(part 1 of 3)
# Autodesk Inventor assembly: Assembly
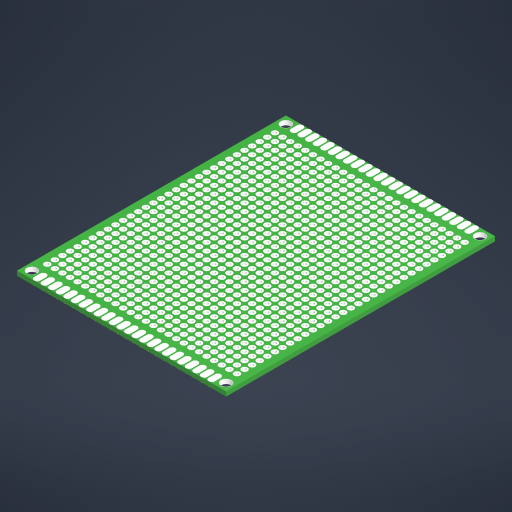
[picture p0: Inventor's stored thumbnail of the model, 512x512]
Saved by Autodesk Inventor 2024 (Build 280153000, 153)
## iProperties
Created: 2024-02-01
Part Number: Assembly
Document SubType Name: Assembly
Designer: Vincent Larson
Title: Universal_board_70x90mm_31x26.stp
Preprocessor: spGate 19.8.4 (****-****-****-****)
## Documents named in this file (908)
- C:\Users\Vincent Larson\Downloads\Universal_board_70x90mm_31x26\Universal_board_70x90mm_31x26.iam
- C:\Users\Vincent Larson\Downloads\Universal_board_70x90mm_31x26\Universal_board_70x90mm_31x26-prt0.ipt
- C:\Users\Vincent Larson\Downloads\Universal_board_70x90mm_31x26\Universal_board_70x90mm_31x26-prt1.ipt
- C:\Users\Vincent Larson\Downloads\Universal_board_70x90mm_31x26\Universal_board_70x90mm_31x26-prt2.ipt
- C:\Users\Vincent Larson\Downloads\Universal_board_70x90mm_31x26\Universal_board_70x90mm_31x26-prt3.ipt
- C:\Users\Vincent Larson\Downloads\Universal_board_70x90mm_31x26\Universal_board_70x90mm_31x26-prt4.ipt
- C:\Users\Vincent Larson\Downloads\Universal_board_70x90mm_31x26\Universal_board_70x90mm_31x26-prt5.ipt
- C:\Users\Vincent Larson\Downloads\Universal_board_70x90mm_31x26\Universal_board_70x90mm_31x26-prt6.ipt
- C:\Users\Vincent Larson\Downloads\Universal_board_70x90mm_31x26\Universal_board_70x90mm_31x26-prt7.ipt
- C:\Users\Vincent Larson\Downloads\Universal_board_70x90mm_31x26\Universal_board_70x90mm_31x26-prt8.ipt
- C:\Users\Vincent Larson\Downloads\Universal_board_70x90mm_31x26\Universal_board_70x90mm_31x26-prt9.ipt
- C:\Users\Vincent Larson\Downloads\Universal_board_70x90mm_31x26\Universal_board_70x90mm_31x26-prt10.ipt
- C:\Users\Vincent Larson\Downloads\Universal_board_70x90mm_31x26\Universal_board_70x90mm_31x26-prt11.ipt
- C:\Users\Vincent Larson\Downloads\Universal_board_70x90mm_31x26\Universal_board_70x90mm_31x26-prt12.ipt
- C:\Users\Vincent Larson\Downloads\Universal_board_70x90mm_31x26\Universal_board_70x90mm_31x26-prt13.ipt
- C:\Users\Vincent Larson\Downloads\Universal_board_70x90mm_31x26\Universal_board_70x90mm_31x26-prt14.ipt
- C:\Users\Vincent Larson\Downloads\Universal_board_70x90mm_31x26\Universal_board_70x90mm_31x26-prt15.ipt
- C:\Users\Vincent Larson\Downloads\Universal_board_70x90mm_31x26\Universal_board_70x90mm_31x26-prt16.ipt
- C:\Users\Vincent Larson\Downloads\Universal_board_70x90mm_31x26\Universal_board_70x90mm_31x26-prt17.ipt
- C:\Users\Vincent Larson\Downloads\Universal_board_70x90mm_31x26\Universal_board_70x90mm_31x26-prt18.ipt
- C:\Users\Vincent Larson\Downloads\Universal_board_70x90mm_31x26\Universal_board_70x90mm_31x26-prt19.ipt
- C:\Users\Vincent Larson\Downloads\Universal_board_70x90mm_31x26\Universal_board_70x90mm_31x26-prt20.ipt
- C:\Users\Vincent Larson\Downloads\Universal_board_70x90mm_31x26\Universal_board_70x90mm_31x26-prt21.ipt
- C:\Users\Vincent Larson\Downloads\Universal_board_70x90mm_31x26\Universal_board_70x90mm_31x26-prt22.ipt
- C:\Users\Vincent Larson\Downloads\Universal_board_70x90mm_31x26\Universal_board_70x90mm_31x26-prt23.ipt
- C:\Users\Vincent Larson\Downloads\Universal_board_70x90mm_31x26\Universal_board_70x90mm_31x26-prt24.ipt
- C:\Users\Vincent Larson\Downloads\Universal_board_70x90mm_31x26\Universal_board_70x90mm_31x26-prt25.ipt
- C:\Users\Vincent Larson\Downloads\Universal_board_70x90mm_31x26\Universal_board_70x90mm_31x26-prt26.ipt
- C:\Users\Vincent Larson\Downloads\Universal_board_70x90mm_31x26\Universal_board_70x90mm_31x26-prt27.ipt
- C:\Users\Vincent Larson\Downloads\Universal_board_70x90mm_31x26\Universal_board_70x90mm_31x26-prt28.ipt
- C:\Users\Vincent Larson\Downloads\Universal_board_70x90mm_31x26\Universal_board_70x90mm_31x26-prt29.ipt
- C:\Users\Vincent Larson\Downloads\Universal_board_70x90mm_31x26\Universal_board_70x90mm_31x26-prt30.ipt
- C:\Users\Vincent Larson\Downloads\Universal_board_70x90mm_31x26\Universal_board_70x90mm_31x26-prt31.ipt
- C:\Users\Vincent Larson\Downloads\Universal_board_70x90mm_31x26\Universal_board_70x90mm_31x26-prt32.ipt
- C:\Users\Vincent Larson\Downloads\Universal_board_70x90mm_31x26\Universal_board_70x90mm_31x26-prt33.ipt
- C:\Users\Vincent Larson\Downloads\Universal_board_70x90mm_31x26\Universal_board_70x90mm_31x26-prt34.ipt
- C:\Users\Vincent Larson\Downloads\Universal_board_70x90mm_31x26\Universal_board_70x90mm_31x26-prt35.ipt
- C:\Users\Vincent Larson\Downloads\Universal_board_70x90mm_31x26\Universal_board_70x90mm_31x26-prt36.ipt
- C:\Users\Vincent Larson\Downloads\Universal_board_70x90mm_31x26\Universal_board_70x90mm_31x26-prt37.ipt
- C:\Users\Vincent Larson\Downloads\Universal_board_70x90mm_31x26\Universal_board_70x90mm_31x26-prt38.ipt
- C:\Users\Vincent Larson\Downloads\Universal_board_70x90mm_31x26\Universal_board_70x90mm_31x26-prt39.ipt
- C:\Users\Vincent Larson\Downloads\Universal_board_70x90mm_31x26\Universal_board_70x90mm_31x26-prt40.ipt
- C:\Users\Vincent Larson\Downloads\Universal_board_70x90mm_31x26\Universal_board_70x90mm_31x26-prt41.ipt
- C:\Users\Vincent Larson\Downloads\Universal_board_70x90mm_31x26\Universal_board_70x90mm_31x26-prt42.ipt
- C:\Users\Vincent Larson\Downloads\Universal_board_70x90mm_31x26\Universal_board_70x90mm_31x26-prt43.ipt
- C:\Users\Vincent Larson\Downloads\Universal_board_70x90mm_31x26\Universal_board_70x90mm_31x26-prt44.ipt
- C:\Users\Vincent Larson\Downloads\Universal_board_70x90mm_31x26\Universal_board_70x90mm_31x26-prt45.ipt
- C:\Users\Vincent Larson\Downloads\Universal_board_70x90mm_31x26\Universal_board_70x90mm_31x26-prt46.ipt
- C:\Users\Vincent Larson\Downloads\Universal_board_70x90mm_31x26\Universal_board_70x90mm_31x26-prt47.ipt
- C:\Users\Vincent Larson\Downloads\Universal_board_70x90mm_31x26\Universal_board_70x90mm_31x26-prt48.ipt
- C:\Users\Vincent Larson\Downloads\Universal_board_70x90mm_31x26\Universal_board_70x90mm_31x26-prt49.ipt
- C:\Users\Vincent Larson\Downloads\Universal_board_70x90mm_31x26\Universal_board_70x90mm_31x26-prt50.ipt
- C:\Users\Vincent Larson\Downloads\Universal_board_70x90mm_31x26\Universal_board_70x90mm_31x26-prt51.ipt
- C:\Users\Vincent Larson\Downloads\Universal_board_70x90mm_31x26\Universal_board_70x90mm_31x26-prt52.ipt
- C:\Users\Vincent Larson\Downloads\Universal_board_70x90mm_31x26\Universal_board_70x90mm_31x26-prt53.ipt
- C:\Users\Vincent Larson\Downloads\Universal_board_70x90mm_31x26\Universal_board_70x90mm_31x26-prt54.ipt
- C:\Users\Vincent Larson\Downloads\Universal_board_70x90mm_31x26\Universal_board_70x90mm_31x26-prt55.ipt
- C:\Users\Vincent Larson\Downloads\Universal_board_70x90mm_31x26\Universal_board_70x90mm_31x26-prt56.ipt
- C:\Users\Vincent Larson\Downloads\Universal_board_70x90mm_31x26\Universal_board_70x90mm_31x26-prt57.ipt
- C:\Users\Vincent Larson\Downloads\Universal_board_70x90mm_31x26\Universal_board_70x90mm_31x26-prt58.ipt
- C:\Users\Vincent Larson\Downloads\Universal_board_70x90mm_31x26\Universal_board_70x90mm_31x26-prt59.ipt
- C:\Users\Vincent Larson\Downloads\Universal_board_70x90mm_31x26\Universal_board_70x90mm_31x26-prt60.ipt
- C:\Users\Vincent Larson\Downloads\Universal_board_70x90mm_31x26\Universal_board_70x90mm_31x26-prt61.ipt
- C:\Users\Vincent Larson\Downloads\Universal_board_70x90mm_31x26\Universal_board_70x90mm_31x26-prt62.ipt
- C:\Users\Vincent Larson\Downloads\Universal_board_70x90mm_31x26\Universal_board_70x90mm_31x26-prt63.ipt
- C:\Users\Vincent Larson\Downloads\Universal_board_70x90mm_31x26\Universal_board_70x90mm_31x26-prt64.ipt
- C:\Users\Vincent Larson\Downloads\Universal_board_70x90mm_31x26\Universal_board_70x90mm_31x26-prt65.ipt
- C:\Users\Vincent Larson\Downloads\Universal_board_70x90mm_31x26\Universal_board_70x90mm_31x26-prt66.ipt
- C:\Users\Vincent Larson\Downloads\Universal_board_70x90mm_31x26\Universal_board_70x90mm_31x26-prt67.ipt
- C:\Users\Vincent Larson\Downloads\Universal_board_70x90mm_31x26\Universal_board_70x90mm_31x26-prt68.ipt
- C:\Users\Vincent Larson\Downloads\Universal_board_70x90mm_31x26\Universal_board_70x90mm_31x26-prt69.ipt
- C:\Users\Vincent Larson\Downloads\Universal_board_70x90mm_31x26\Universal_board_70x90mm_31x26-prt70.ipt
- C:\Users\Vincent Larson\Downloads\Universal_board_70x90mm_31x26\Universal_board_70x90mm_31x26-prt71.ipt
- C:\Users\Vincent Larson\Downloads\Universal_board_70x90mm_31x26\Universal_board_70x90mm_31x26-prt72.ipt
- C:\Users\Vincent Larson\Downloads\Universal_board_70x90mm_31x26\Universal_board_70x90mm_31x26-prt73.ipt
- C:\Users\Vincent Larson\Downloads\Universal_board_70x90mm_31x26\Universal_board_70x90mm_31x26-prt74.ipt
- C:\Users\Vincent Larson\Downloads\Universal_board_70x90mm_31x26\Universal_board_70x90mm_31x26-prt75.ipt
- C:\Users\Vincent Larson\Downloads\Universal_board_70x90mm_31x26\Universal_board_70x90mm_31x26-prt76.ipt
- C:\Users\Vincent Larson\Downloads\Universal_board_70x90mm_31x26\Universal_board_70x90mm_31x26-prt77.ipt
- C:\Users\Vincent Larson\Downloads\Universal_board_70x90mm_31x26\Universal_board_70x90mm_31x26-prt78.ipt
- C:\Users\Vincent Larson\Downloads\Universal_board_70x90mm_31x26\Universal_board_70x90mm_31x26-prt79.ipt
- C:\Users\Vincent Larson\Downloads\Universal_board_70x90mm_31x26\Universal_board_70x90mm_31x26-prt80.ipt
- C:\Users\Vincent Larson\Downloads\Universal_board_70x90mm_31x26\Universal_board_70x90mm_31x26-prt81.ipt
- C:\Users\Vincent Larson\Downloads\Universal_board_70x90mm_31x26\Universal_board_70x90mm_31x26-prt82.ipt
- C:\Users\Vincent Larson\Downloads\Universal_board_70x90mm_31x26\Universal_board_70x90mm_31x26-prt83.ipt
- C:\Users\Vincent Larson\Downloads\Universal_board_70x90mm_31x26\Universal_board_70x90mm_31x26-prt84.ipt
- C:\Users\Vincent Larson\Downloads\Universal_board_70x90mm_31x26\Universal_board_70x90mm_31x26-prt85.ipt
- C:\Users\Vincent Larson\Downloads\Universal_board_70x90mm_31x26\Universal_board_70x90mm_31x26-prt86.ipt
- C:\Users\Vincent Larson\Downloads\Universal_board_70x90mm_31x26\Universal_board_70x90mm_31x26-prt87.ipt
- C:\Users\Vincent Larson\Downloads\Universal_board_70x90mm_31x26\Universal_board_70x90mm_31x26-prt88.ipt
- C:\Users\Vincent Larson\Downloads\Universal_board_70x90mm_31x26\Universal_board_70x90mm_31x26-prt89.ipt
- C:\Users\Vincent Larson\Downloads\Universal_board_70x90mm_31x26\Universal_board_70x90mm_31x26-prt90.ipt
- C:\Users\Vincent Larson\Downloads\Universal_board_70x90mm_31x26\Universal_board_70x90mm_31x26-prt91.ipt
- C:\Users\Vincent Larson\Downloads\Universal_board_70x90mm_31x26\Universal_board_70x90mm_31x26-prt92.ipt
- C:\Users\Vincent Larson\Downloads\Universal_board_70x90mm_31x26\Universal_board_70x90mm_31x26-prt93.ipt
- C:\Users\Vincent Larson\Downloads\Universal_board_70x90mm_31x26\Universal_board_70x90mm_31x26-prt94.ipt
- C:\Users\Vincent Larson\Downloads\Universal_board_70x90mm_31x26\Universal_board_70x90mm_31x26-prt95.ipt
- C:\Users\Vincent Larson\Downloads\Universal_board_70x90mm_31x26\Universal_board_70x90mm_31x26-prt96.ipt
- C:\Users\Vincent Larson\Downloads\Universal_board_70x90mm_31x26\Universal_board_70x90mm_31x26-prt97.ipt
- C:\Users\Vincent Larson\Downloads\Universal_board_70x90mm_31x26\Universal_board_70x90mm_31x26-prt98.ipt
- C:\Users\Vincent Larson\Downloads\Universal_board_70x90mm_31x26\Universal_board_70x90mm_31x26-prt99.ipt
- C:\Users\Vincent Larson\Downloads\Universal_board_70x90mm_31x26\Universal_board_70x90mm_31x26-prt100.ipt
- C:\Users\Vincent Larson\Downloads\Universal_board_70x90mm_31x26\Universal_board_70x90mm_31x26-prt101.ipt
- C:\Users\Vincent Larson\Downloads\Universal_board_70x90mm_31x26\Universal_board_70x90mm_31x26-prt102.ipt
- C:\Users\Vincent Larson\Downloads\Universal_board_70x90mm_31x26\Universal_board_70x90mm_31x26-prt103.ipt
- C:\Users\Vincent Larson\Downloads\Universal_board_70x90mm_31x26\Universal_board_70x90mm_31x26-prt104.ipt
- C:\Users\Vincent Larson\Downloads\Universal_board_70x90mm_31x26\Universal_board_70x90mm_31x26-prt105.ipt
- C:\Users\Vincent Larson\Downloads\Universal_board_70x90mm_31x26\Universal_board_70x90mm_31x26-prt106.ipt
- C:\Users\Vincent Larson\Downloads\Universal_board_70x90mm_31x26\Universal_board_70x90mm_31x26-prt107.ipt
- C:\Users\Vincent Larson\Downloads\Universal_board_70x90mm_31x26\Universal_board_70x90mm_31x26-prt108.ipt
- C:\Users\Vincent Larson\Downloads\Universal_board_70x90mm_31x26\Universal_board_70x90mm_31x26-prt109.ipt
- C:\Users\Vincent Larson\Downloads\Universal_board_70x90mm_31x26\Universal_board_70x90mm_31x26-prt110.ipt
- C:\Users\Vincent Larson\Downloads\Universal_board_70x90mm_31x26\Universal_board_70x90mm_31x26-prt111.ipt
- C:\Users\Vincent Larson\Downloads\Universal_board_70x90mm_31x26\Universal_board_70x90mm_31x26-prt112.ipt
- C:\Users\Vincent Larson\Downloads\Universal_board_70x90mm_31x26\Universal_board_70x90mm_31x26-prt113.ipt
- C:\Users\Vincent Larson\Downloads\Universal_board_70x90mm_31x26\Universal_board_70x90mm_31x26-prt114.ipt
- C:\Users\Vincent Larson\Downloads\Universal_board_70x90mm_31x26\Universal_board_70x90mm_31x26-prt115.ipt
- C:\Users\Vincent Larson\Downloads\Universal_board_70x90mm_31x26\Universal_board_70x90mm_31x26-prt116.ipt
- C:\Users\Vincent Larson\Downloads\Universal_board_70x90mm_31x26\Universal_board_70x90mm_31x26-prt117.ipt
- C:\Users\Vincent Larson\Downloads\Universal_board_70x90mm_31x26\Universal_board_70x90mm_31x26-prt118.ipt
- C:\Users\Vincent Larson\Downloads\Universal_board_70x90mm_31x26\Universal_board_70x90mm_31x26-prt119.ipt
- C:\Users\Vincent Larson\Downloads\Universal_board_70x90mm_31x26\Universal_board_70x90mm_31x26-prt120.ipt
- C:\Users\Vincent Larson\Downloads\Universal_board_70x90mm_31x26\Universal_board_70x90mm_31x26-prt121.ipt
- C:\Users\Vincent Larson\Downloads\Universal_board_70x90mm_31x26\Universal_board_70x90mm_31x26-prt122.ipt
- C:\Users\Vincent Larson\Downloads\Universal_board_70x90mm_31x26\Universal_board_70x90mm_31x26-prt123.ipt
- C:\Users\Vincent Larson\Downloads\Universal_board_70x90mm_31x26\Universal_board_70x90mm_31x26-prt124.ipt
- C:\Users\Vincent Larson\Downloads\Universal_board_70x90mm_31x26\Universal_board_70x90mm_31x26-prt125.ipt
- C:\Users\Vincent Larson\Downloads\Universal_board_70x90mm_31x26\Universal_board_70x90mm_31x26-prt126.ipt
- C:\Users\Vincent Larson\Downloads\Universal_board_70x90mm_31x26\Universal_board_70x90mm_31x26-prt127.ipt
- C:\Users\Vincent Larson\Downloads\Universal_board_70x90mm_31x26\Universal_board_70x90mm_31x26-prt128.ipt
- C:\Users\Vincent Larson\Downloads\Universal_board_70x90mm_31x26\Universal_board_70x90mm_31x26-prt129.ipt
- C:\Users\Vincent Larson\Downloads\Universal_board_70x90mm_31x26\Universal_board_70x90mm_31x26-prt130.ipt
- C:\Users\Vincent Larson\Downloads\Universal_board_70x90mm_31x26\Universal_board_70x90mm_31x26-prt131.ipt
- C:\Users\Vincent Larson\Downloads\Universal_board_70x90mm_31x26\Universal_board_70x90mm_31x26-prt132.ipt
- C:\Users\Vincent Larson\Downloads\Universal_board_70x90mm_31x26\Universal_board_70x90mm_31x26-prt133.ipt
- C:\Users\Vincent Larson\Downloads\Universal_board_70x90mm_31x26\Universal_board_70x90mm_31x26-prt134.ipt
- C:\Users\Vincent Larson\Downloads\Universal_board_70x90mm_31x26\Universal_board_70x90mm_31x26-prt135.ipt
- C:\Users\Vincent Larson\Downloads\Universal_board_70x90mm_31x26\Universal_board_70x90mm_31x26-prt136.ipt
- C:\Users\Vincent Larson\Downloads\Universal_board_70x90mm_31x26\Universal_board_70x90mm_31x26-prt137.ipt
- C:\Users\Vincent Larson\Downloads\Universal_board_70x90mm_31x26\Universal_board_70x90mm_31x26-prt138.ipt
- C:\Users\Vincent Larson\Downloads\Universal_board_70x90mm_31x26\Universal_board_70x90mm_31x26-prt139.ipt
- C:\Users\Vincent Larson\Downloads\Universal_board_70x90mm_31x26\Universal_board_70x90mm_31x26-prt140.ipt
- C:\Users\Vincent Larson\Downloads\Universal_board_70x90mm_31x26\Universal_board_70x90mm_31x26-prt141.ipt
- C:\Users\Vincent Larson\Downloads\Universal_board_70x90mm_31x26\Universal_board_70x90mm_31x26-prt142.ipt
- C:\Users\Vincent Larson\Downloads\Universal_board_70x90mm_31x26\Universal_board_70x90mm_31x26-prt143.ipt
- C:\Users\Vincent Larson\Downloads\Universal_board_70x90mm_31x26\Universal_board_70x90mm_31x26-prt144.ipt
- C:\Users\Vincent Larson\Downloads\Universal_board_70x90mm_31x26\Universal_board_70x90mm_31x26-prt145.ipt
- C:\Users\Vincent Larson\Downloads\Universal_board_70x90mm_31x26\Universal_board_70x90mm_31x26-prt146.ipt
- C:\Users\Vincent Larson\Downloads\Universal_board_70x90mm_31x26\Universal_board_70x90mm_31x26-prt147.ipt
- C:\Users\Vincent Larson\Downloads\Universal_board_70x90mm_31x26\Universal_board_70x90mm_31x26-prt148.ipt
- C:\Users\Vincent Larson\Downloads\Universal_board_70x90mm_31x26\Universal_board_70x90mm_31x26-prt149.ipt
- C:\Users\Vincent Larson\Downloads\Universal_board_70x90mm_31x26\Universal_board_70x90mm_31x26-prt150.ipt
- C:\Users\Vincent Larson\Downloads\Universal_board_70x90mm_31x26\Universal_board_70x90mm_31x26-prt151.ipt
- C:\Users\Vincent Larson\Downloads\Universal_board_70x90mm_31x26\Universal_board_70x90mm_31x26-prt152.ipt
- C:\Users\Vincent Larson\Downloads\Universal_board_70x90mm_31x26\Universal_board_70x90mm_31x26-prt153.ipt
- C:\Users\Vincent Larson\Downloads\Universal_board_70x90mm_31x26\Universal_board_70x90mm_31x26-prt154.ipt
- C:\Users\Vincent Larson\Downloads\Universal_board_70x90mm_31x26\Universal_board_70x90mm_31x26-prt155.ipt
- C:\Users\Vincent Larson\Downloads\Universal_board_70x90mm_31x26\Universal_board_70x90mm_31x26-prt156.ipt
- C:\Users\Vincent Larson\Downloads\Universal_board_70x90mm_31x26\Universal_board_70x90mm_31x26-prt157.ipt
- C:\Users\Vincent Larson\Downloads\Universal_board_70x90mm_31x26\Universal_board_70x90mm_31x26-prt158.ipt
- C:\Users\Vincent Larson\Downloads\Universal_board_70x90mm_31x26\Universal_board_70x90mm_31x26-prt159.ipt
- C:\Users\Vincent Larson\Downloads\Universal_board_70x90mm_31x26\Universal_board_70x90mm_31x26-prt160.ipt
- C:\Users\Vincent Larson\Downloads\Universal_board_70x90mm_31x26\Universal_board_70x90mm_31x26-prt161.ipt
- C:\Users\Vincent Larson\Downloads\Universal_board_70x90mm_31x26\Universal_board_70x90mm_31x26-prt162.ipt
- C:\Users\Vincent Larson\Downloads\Universal_board_70x90mm_31x26\Universal_board_70x90mm_31x26-prt163.ipt
- C:\Users\Vincent Larson\Downloads\Universal_board_70x90mm_31x26\Universal_board_70x90mm_31x26-prt164.ipt
- C:\Users\Vincent Larson\Downloads\Universal_board_70x90mm_31x26\Universal_board_70x90mm_31x26-prt165.ipt
- C:\Users\Vincent Larson\Downloads\Universal_board_70x90mm_31x26\Universal_board_70x90mm_31x26-prt166.ipt
- C:\Users\Vincent Larson\Downloads\Universal_board_70x90mm_31x26\Universal_board_70x90mm_31x26-prt167.ipt
- C:\Users\Vincent Larson\Downloads\Universal_board_70x90mm_31x26\Universal_board_70x90mm_31x26-prt168.ipt
- C:\Users\Vincent Larson\Downloads\Universal_board_70x90mm_31x26\Universal_board_70x90mm_31x26-prt169.ipt
- C:\Users\Vincent Larson\Downloads\Universal_board_70x90mm_31x26\Universal_board_70x90mm_31x26-prt170.ipt
- C:\Users\Vincent Larson\Downloads\Universal_board_70x90mm_31x26\Universal_board_70x90mm_31x26-prt171.ipt
- C:\Users\Vincent Larson\Downloads\Universal_board_70x90mm_31x26\Universal_board_70x90mm_31x26-prt172.ipt
- C:\Users\Vincent Larson\Downloads\Universal_board_70x90mm_31x26\Universal_board_70x90mm_31x26-prt173.ipt
- C:\Users\Vincent Larson\Downloads\Universal_board_70x90mm_31x26\Universal_board_70x90mm_31x26-prt174.ipt
- C:\Users\Vincent Larson\Downloads\Universal_board_70x90mm_31x26\Universal_board_70x90mm_31x26-prt175.ipt
- C:\Users\Vincent Larson\Downloads\Universal_board_70x90mm_31x26\Universal_board_70x90mm_31x26-prt176.ipt
- C:\Users\Vincent Larson\Downloads\Universal_board_70x90mm_31x26\Universal_board_70x90mm_31x26-prt177.ipt
- C:\Users\Vincent Larson\Downloads\Universal_board_70x90mm_31x26\Universal_board_70x90mm_31x26-prt178.ipt
- C:\Users\Vincent Larson\Downloads\Universal_board_70x90mm_31x26\Universal_board_70x90mm_31x26-prt179.ipt
- C:\Users\Vincent Larson\Downloads\Universal_board_70x90mm_31x26\Universal_board_70x90mm_31x26-prt180.ipt
- C:\Users\Vincent Larson\Downloads\Universal_board_70x90mm_31x26\Universal_board_70x90mm_31x26-prt181.ipt
- C:\Users\Vincent Larson\Downloads\Universal_board_70x90mm_31x26\Universal_board_70x90mm_31x26-prt182.ipt
- C:\Users\Vincent Larson\Downloads\Universal_board_70x90mm_31x26\Universal_board_70x90mm_31x26-prt183.ipt
- C:\Users\Vincent Larson\Downloads\Universal_board_70x90mm_31x26\Universal_board_70x90mm_31x26-prt184.ipt
- C:\Users\Vincent Larson\Downloads\Universal_board_70x90mm_31x26\Universal_board_70x90mm_31x26-prt185.ipt
- C:\Users\Vincent Larson\Downloads\Universal_board_70x90mm_31x26\Universal_board_70x90mm_31x26-prt186.ipt
- C:\Users\Vincent Larson\Downloads\Universal_board_70x90mm_31x26\Universal_board_70x90mm_31x26-prt187.ipt
- C:\Users\Vincent Larson\Downloads\Universal_board_70x90mm_31x26\Universal_board_70x90mm_31x26-prt188.ipt
- C:\Users\Vincent Larson\Downloads\Universal_board_70x90mm_31x26\Universal_board_70x90mm_31x26-prt189.ipt
- C:\Users\Vincent Larson\Downloads\Universal_board_70x90mm_31x26\Universal_board_70x90mm_31x26-prt190.ipt
- C:\Users\Vincent Larson\Downloads\Universal_board_70x90mm_31x26\Universal_board_70x90mm_31x26-prt191.ipt
- C:\Users\Vincent Larson\Downloads\Universal_board_70x90mm_31x26\Universal_board_70x90mm_31x26-prt192.ipt
- C:\Users\Vincent Larson\Downloads\Universal_board_70x90mm_31x26\Universal_board_70x90mm_31x26-prt193.ipt
- C:\Users\Vincent Larson\Downloads\Universal_board_70x90mm_31x26\Universal_board_70x90mm_31x26-prt194.ipt
- C:\Users\Vincent Larson\Downloads\Universal_board_70x90mm_31x26\Universal_board_70x90mm_31x26-prt195.ipt
- C:\Users\Vincent Larson\Downloads\Universal_board_70x90mm_31x26\Universal_board_70x90mm_31x26-prt196.ipt
- C:\Users\Vincent Larson\Downloads\Universal_board_70x90mm_31x26\Universal_board_70x90mm_31x26-prt197.ipt
- C:\Users\Vincent Larson\Downloads\Universal_board_70x90mm_31x26\Universal_board_70x90mm_31x26-prt198.ipt
- C:\Users\Vincent Larson\Downloads\Universal_board_70x90mm_31x26\Universal_board_70x90mm_31x26-prt199.ipt
- C:\Users\Vincent Larson\Downloads\Universal_board_70x90mm_31x26\Universal_board_70x90mm_31x26-prt200.ipt
- C:\Users\Vincent Larson\Downloads\Universal_board_70x90mm_31x26\Universal_board_70x90mm_31x26-prt201.ipt
- C:\Users\Vincent Larson\Downloads\Universal_board_70x90mm_31x26\Universal_board_70x90mm_31x26-prt202.ipt
- C:\Users\Vincent Larson\Downloads\Universal_board_70x90mm_31x26\Universal_board_70x90mm_31x26-prt203.ipt
- C:\Users\Vincent Larson\Downloads\Universal_board_70x90mm_31x26\Universal_board_70x90mm_31x26-prt204.ipt
- C:\Users\Vincent Larson\Downloads\Universal_board_70x90mm_31x26\Universal_board_70x90mm_31x26-prt205.ipt
- C:\Users\Vincent Larson\Downloads\Universal_board_70x90mm_31x26\Universal_board_70x90mm_31x26-prt206.ipt
- C:\Users\Vincent Larson\Downloads\Universal_board_70x90mm_31x26\Universal_board_70x90mm_31x26-prt207.ipt
- C:\Users\Vincent Larson\Downloads\Universal_board_70x90mm_31x26\Universal_board_70x90mm_31x26-prt208.ipt
- C:\Users\Vincent Larson\Downloads\Universal_board_70x90mm_31x26\Universal_board_70x90mm_31x26-prt209.ipt
- C:\Users\Vincent Larson\Downloads\Universal_board_70x90mm_31x26\Universal_board_70x90mm_31x26-prt210.ipt
- C:\Users\Vincent Larson\Downloads\Universal_board_70x90mm_31x26\Universal_board_70x90mm_31x26-prt211.ipt
- C:\Users\Vincent Larson\Downloads\Universal_board_70x90mm_31x26\Universal_board_70x90mm_31x26-prt212.ipt
- C:\Users\Vincent Larson\Downloads\Universal_board_70x90mm_31x26\Universal_board_70x90mm_31x26-prt213.ipt
- C:\Users\Vincent Larson\Downloads\Universal_board_70x90mm_31x26\Universal_board_70x90mm_31x26-prt214.ipt
- C:\Users\Vincent Larson\Downloads\Universal_board_70x90mm_31x26\Universal_board_70x90mm_31x26-prt215.ipt
- C:\Users\Vincent Larson\Downloads\Universal_board_70x90mm_31x26\Universal_board_70x90mm_31x26-prt216.ipt
- C:\Users\Vincent Larson\Downloads\Universal_board_70x90mm_31x26\Universal_board_70x90mm_31x26-prt217.ipt
- C:\Users\Vincent Larson\Downloads\Universal_board_70x90mm_31x26\Universal_board_70x90mm_31x26-prt218.ipt
- C:\Users\Vincent Larson\Downloads\Universal_board_70x90mm_31x26\Universal_board_70x90mm_31x26-prt219.ipt
- C:\Users\Vincent Larson\Downloads\Universal_board_70x90mm_31x26\Universal_board_70x90mm_31x26-prt220.ipt
- C:\Users\Vincent Larson\Downloads\Universal_board_70x90mm_31x26\Universal_board_70x90mm_31x26-prt221.ipt
- C:\Users\Vincent Larson\Downloads\Universal_board_70x90mm_31x26\Universal_board_70x90mm_31x26-prt222.ipt
- C:\Users\Vincent Larson\Downloads\Universal_board_70x90mm_31x26\Universal_board_70x90mm_31x26-prt223.ipt
- C:\Users\Vincent Larson\Downloads\Universal_board_70x90mm_31x26\Universal_board_70x90mm_31x26-prt224.ipt
- C:\Users\Vincent Larson\Downloads\Universal_board_70x90mm_31x26\Universal_board_70x90mm_31x26-prt225.ipt
- C:\Users\Vincent Larson\Downloads\Universal_board_70x90mm_31x26\Universal_board_70x90mm_31x26-prt226.ipt
- C:\Users\Vincent Larson\Downloads\Universal_board_70x90mm_31x26\Universal_board_70x90mm_31x26-prt227.ipt
- C:\Users\Vincent Larson\Downloads\Universal_board_70x90mm_31x26\Universal_board_70x90mm_31x26-prt228.ipt
- C:\Users\Vincent Larson\Downloads\Universal_board_70x90mm_31x26\Universal_board_70x90mm_31x26-prt229.ipt
- C:\Users\Vincent Larson\Downloads\Universal_board_70x90mm_31x26\Universal_board_70x90mm_31x26-prt230.ipt
- C:\Users\Vincent Larson\Downloads\Universal_board_70x90mm_31x26\Universal_board_70x90mm_31x26-prt231.ipt
- C:\Users\Vincent Larson\Downloads\Universal_board_70x90mm_31x26\Universal_board_70x90mm_31x26-prt232.ipt
- C:\Users\Vincent Larson\Downloads\Universal_board_70x90mm_31x26\Universal_board_70x90mm_31x26-prt233.ipt
- C:\Users\Vincent Larson\Downloads\Universal_board_70x90mm_31x26\Universal_board_70x90mm_31x26-prt234.ipt
- C:\Users\Vincent Larson\Downloads\Universal_board_70x90mm_31x26\Universal_board_70x90mm_31x26-prt235.ipt
- C:\Users\Vincent Larson\Downloads\Universal_board_70x90mm_31x26\Universal_board_70x90mm_31x26-prt236.ipt
- C:\Users\Vincent Larson\Downloads\Universal_board_70x90mm_31x26\Universal_board_70x90mm_31x26-prt237.ipt
- C:\Users\Vincent Larson\Downloads\Universal_board_70x90mm_31x26\Universal_board_70x90mm_31x26-prt238.ipt
- C:\Users\Vincent Larson\Downloads\Universal_board_70x90mm_31x26\Universal_board_70x90mm_31x26-prt239.ipt
- C:\Users\Vincent Larson\Downloads\Universal_board_70x90mm_31x26\Universal_board_70x90mm_31x26-prt240.ipt
- C:\Users\Vincent Larson\Downloads\Universal_board_70x90mm_31x26\Universal_board_70x90mm_31x26-prt241.ipt
- C:\Users\Vincent Larson\Downloads\Universal_board_70x90mm_31x26\Universal_board_70x90mm_31x26-prt242.ipt
- C:\Users\Vincent Larson\Downloads\Universal_board_70x90mm_31x26\Universal_board_70x90mm_31x26-prt243.ipt
- C:\Users\Vincent Larson\Downloads\Universal_board_70x90mm_31x26\Universal_board_70x90mm_31x26-prt244.ipt
- C:\Users\Vincent Larson\Downloads\Universal_board_70x90mm_31x26\Universal_board_70x90mm_31x26-prt245.ipt
- C:\Users\Vincent Larson\Downloads\Universal_board_70x90mm_31x26\Universal_board_70x90mm_31x26-prt246.ipt
- C:\Users\Vincent Larson\Downloads\Universal_board_70x90mm_31x26\Universal_board_70x90mm_31x26-prt247.ipt
- C:\Users\Vincent Larson\Downloads\Universal_board_70x90mm_31x26\Universal_board_70x90mm_31x26-prt248.ipt
- C:\Users\Vincent Larson\Downloads\Universal_board_70x90mm_31x26\Universal_board_70x90mm_31x26-prt249.ipt
- C:\Users\Vincent Larson\Downloads\Universal_board_70x90mm_31x26\Universal_board_70x90mm_31x26-prt250.ipt
- C:\Users\Vincent Larson\Downloads\Universal_board_70x90mm_31x26\Universal_board_70x90mm_31x26-prt251.ipt
- C:\Users\Vincent Larson\Downloads\Universal_board_70x90mm_31x26\Universal_board_70x90mm_31x26-prt252.ipt
- C:\Users\Vincent Larson\Downloads\Universal_board_70x90mm_31x26\Universal_board_70x90mm_31x26-prt253.ipt
- C:\Users\Vincent Larson\Downloads\Universal_board_70x90mm_31x26\Universal_board_70x90mm_31x26-prt254.ipt
- C:\Users\Vincent Larson\Downloads\Universal_board_70x90mm_31x26\Universal_board_70x90mm_31x26-prt255.ipt
- C:\Users\Vincent Larson\Downloads\Universal_board_70x90mm_31x26\Universal_board_70x90mm_31x26-prt256.ipt
- C:\Users\Vincent Larson\Downloads\Universal_board_70x90mm_31x26\Universal_board_70x90mm_31x26-prt257.ipt
- C:\Users\Vincent Larson\Downloads\Universal_board_70x90mm_31x26\Universal_board_70x90mm_31x26-prt258.ipt
- C:\Users\Vincent Larson\Downloads\Universal_board_70x90mm_31x26\Universal_board_70x90mm_31x26-prt259.ipt
- C:\Users\Vincent Larson\Downloads\Universal_board_70x90mm_31x26\Universal_board_70x90mm_31x26-prt260.ipt
- C:\Users\Vincent Larson\Downloads\Universal_board_70x90mm_31x26\Universal_board_70x90mm_31x26-prt261.ipt
- C:\Users\Vincent Larson\Downloads\Universal_board_70x90mm_31x26\Universal_board_70x90mm_31x26-prt262.ipt
- C:\Users\Vincent Larson\Downloads\Universal_board_70x90mm_31x26\Universal_board_70x90mm_31x26-prt263.ipt
- C:\Users\Vincent Larson\Downloads\Universal_board_70x90mm_31x26\Universal_board_70x90mm_31x26-prt264.ipt
- C:\Users\Vincent Larson\Downloads\Universal_board_70x90mm_31x26\Universal_board_70x90mm_31x26-prt265.ipt
- C:\Users\Vincent Larson\Downloads\Universal_board_70x90mm_31x26\Universal_board_70x90mm_31x26-prt266.ipt
- C:\Users\Vincent Larson\Downloads\Universal_board_70x90mm_31x26\Universal_board_70x90mm_31x26-prt267.ipt
- C:\Users\Vincent Larson\Downloads\Universal_board_70x90mm_31x26\Universal_board_70x90mm_31x26-prt268.ipt
- C:\Users\Vincent Larson\Downloads\Universal_board_70x90mm_31x26\Universal_board_70x90mm_31x26-prt269.ipt
- C:\Users\Vincent Larson\Downloads\Universal_board_70x90mm_31x26\Universal_board_70x90mm_31x26-prt270.ipt
- C:\Users\Vincent Larson\Downloads\Universal_board_70x90mm_31x26\Universal_board_70x90mm_31x26-prt271.ipt
- C:\Users\Vincent Larson\Downloads\Universal_board_70x90mm_31x26\Universal_board_70x90mm_31x26-prt272.ipt
- C:\Users\Vincent Larson\Downloads\Universal_board_70x90mm_31x26\Universal_board_70x90mm_31x26-prt273.ipt
- C:\Users\Vincent Larson\Downloads\Universal_board_70x90mm_31x26\Universal_board_70x90mm_31x26-prt274.ipt
- C:\Users\Vincent Larson\Downloads\Universal_board_70x90mm_31x26\Universal_board_70x90mm_31x26-prt275.ipt
- C:\Users\Vincent Larson\Downloads\Universal_board_70x90mm_31x26\Universal_board_70x90mm_31x26-prt276.ipt
- C:\Users\Vincent Larson\Downloads\Universal_board_70x90mm_31x26\Universal_board_70x90mm_31x26-prt277.ipt
- C:\Users\Vincent Larson\Downloads\Universal_board_70x90mm_31x26\Universal_board_70x90mm_31x26-prt278.ipt
- C:\Users\Vincent Larson\Downloads\Universal_board_70x90mm_31x26\Universal_board_70x90mm_31x26-prt279.ipt
- C:\Users\Vincent Larson\Downloads\Universal_board_70x90mm_31x26\Universal_board_70x90mm_31x26-prt280.ipt
- C:\Users\Vincent Larson\Downloads\Universal_board_70x90mm_31x26\Universal_board_70x90mm_31x26-prt281.ipt
- C:\Users\Vincent Larson\Downloads\Universal_board_70x90mm_31x26\Universal_board_70x90mm_31x26-prt282.ipt
- C:\Users\Vincent Larson\Downloads\Universal_board_70x90mm_31x26\Universal_board_70x90mm_31x26-prt283.ipt
- C:\Users\Vincent Larson\Downloads\Universal_board_70x90mm_31x26\Universal_board_70x90mm_31x26-prt284.ipt
- C:\Users\Vincent Larson\Downloads\Universal_board_70x90mm_31x26\Universal_board_70x90mm_31x26-prt285.ipt
- C:\Users\Vincent Larson\Downloads\Universal_board_70x90mm_31x26\Universal_board_70x90mm_31x26-prt286.ipt
- C:\Users\Vincent Larson\Downloads\Universal_board_70x90mm_31x26\Universal_board_70x90mm_31x26-prt287.ipt
- C:\Users\Vincent Larson\Downloads\Universal_board_70x90mm_31x26\Universal_board_70x90mm_31x26-prt288.ipt
- C:\Users\Vincent Larson\Downloads\Universal_board_70x90mm_31x26\Universal_board_70x90mm_31x26-prt289.ipt
- C:\Users\Vincent Larson\Downloads\Universal_board_70x90mm_31x26\Universal_board_70x90mm_31x26-prt290.ipt
- C:\Users\Vincent Larson\Downloads\Universal_board_70x90mm_31x26\Universal_board_70x90mm_31x26-prt291.ipt
- C:\Users\Vincent Larson\Downloads\Universal_board_70x90mm_31x26\Universal_board_70x90mm_31x26-prt292.ipt
- C:\Users\Vincent Larson\Downloads\Universal_board_70x90mm_31x26\Universal_board_70x90mm_31x26-prt293.ipt
- C:\Users\Vincent Larson\Downloads\Universal_board_70x90mm_31x26\Universal_board_70x90mm_31x26-prt294.ipt
- C:\Users\Vincent Larson\Downloads\Universal_board_70x90mm_31x26\Universal_board_70x90mm_31x26-prt295.ipt
- C:\Users\Vincent Larson\Downloads\Universal_board_70x90mm_31x26\Universal_board_70x90mm_31x26-prt296.ipt
- C:\Users\Vincent Larson\Downloads\Universal_board_70x90mm_31x26\Universal_board_70x90mm_31x26-prt297.ipt
- C:\Users\Vincent Larson\Downloads\Universal_board_70x90mm_31x26\Universal_board_70x90mm_31x26-prt298.ipt
- C:\Users\Vincent Larson\Downloads\Universal_board_70x90mm_31x26\Universal_board_70x90mm_31x26-prt299.ipt
- C:\Users\Vincent Larson\Downloads\Universal_board_70x90mm_31x26\Universal_board_70x90mm_31x26-prt300.ipt
- C:\Users\Vincent Larson\Downloads\Universal_board_70x90mm_31x26\Universal_board_70x90mm_31x26-prt301.ipt
- C:\Users\Vincent Larson\Downloads\Universal_board_70x90mm_31x26\Universal_board_70x90mm_31x26-prt302.ipt
- C:\Users\Vincent Larson\Downloads\Universal_board_70x90mm_31x26\Universal_board_70x90mm_31x26-prt303.ipt
- C:\Users\Vincent Larson\Downloads\Universal_board_70x90mm_31x26\Universal_board_70x90mm_31x26-prt304.ipt
- C:\Users\Vincent Larson\Downloads\Universal_board_70x90mm_31x26\Universal_board_70x90mm_31x26-prt305.ipt
- C:\Users\Vincent Larson\Downloads\Universal_board_70x90mm_31x26\Universal_board_70x90mm_31x26-prt306.ipt
- C:\Users\Vincent Larson\Downloads\Universal_board_70x90mm_31x26\Universal_board_70x90mm_31x26-prt307.ipt
- C:\Users\Vincent Larson\Downloads\Universal_board_70x90mm_31x26\Universal_board_70x90mm_31x26-prt308.ipt
- C:\Users\Vincent Larson\Downloads\Universal_board_70x90mm_31x26\Universal_board_70x90mm_31x26-prt309.ipt
- C:\Users\Vincent Larson\Downloads\Universal_board_70x90mm_31x26\Universal_board_70x90mm_31x26-prt310.ipt
- C:\Users\Vincent Larson\Downloads\Universal_board_70x90mm_31x26\Universal_board_70x90mm_31x26-prt311.ipt
- C:\Users\Vincent Larson\Downloads\Universal_board_70x90mm_31x26\Universal_board_70x90mm_31x26-prt312.ipt
- C:\Users\Vincent Larson\Downloads\Universal_board_70x90mm_31x26\Universal_board_70x90mm_31x26-prt313.ipt
- C:\Users\Vincent Larson\Downloads\Universal_board_70x90mm_31x26\Universal_board_70x90mm_31x26-prt314.ipt
- C:\Users\Vincent Larson\Downloads\Universal_board_70x90mm_31x26\Universal_board_70x90mm_31x26-prt315.ipt
- C:\Users\Vincent Larson\Downloads\Universal_board_70x90mm_31x26\Universal_board_70x90mm_31x26-prt316.ipt
- C:\Users\Vincent Larson\Downloads\Universal_board_70x90mm_31x26\Universal_board_70x90mm_31x26-prt317.ipt
- C:\Users\Vincent Larson\Downloads\Universal_board_70x90mm_31x26\Universal_board_70x90mm_31x26-prt318.ipt
- C:\Users\Vincent Larson\Downloads\Universal_board_70x90mm_31x26\Universal_board_70x90mm_31x26-prt319.ipt
- C:\Users\Vincent Larson\Downloads\Universal_board_70x90mm_31x26\Universal_board_70x90mm_31x26-prt320.ipt
- C:\Users\Vincent Larson\Downloads\Universal_board_70x90mm_31x26\Universal_board_70x90mm_31x26-prt321.ipt
- C:\Users\Vincent Larson\Downloads\Universal_board_70x90mm_31x26\Universal_board_70x90mm_31x26-prt322.ipt
- C:\Users\Vincent Larson\Downloads\Universal_board_70x90mm_31x26\Universal_board_70x90mm_31x26-prt323.ipt
- C:\Users\Vincent Larson\Downloads\Universal_board_70x90mm_31x26\Universal_board_70x90mm_31x26-prt324.ipt
- C:\Users\Vincent Larson\Downloads\Universal_board_70x90mm_31x26\Universal_board_70x90mm_31x26-prt325.ipt
- C:\Users\Vincent Larson\Downloads\Universal_board_70x90mm_31x26\Universal_board_70x90mm_31x26-prt326.ipt
- C:\Users\Vincent Larson\Downloads\Universal_board_70x90mm_31x26\Universal_board_70x90mm_31x26-prt327.ipt
- C:\Users\Vincent Larson\Downloads\Universal_board_70x90mm_31x26\Universal_board_70x90mm_31x26-prt328.ipt
- C:\Users\Vincent Larson\Downloads\Universal_board_70x90mm_31x26\Universal_board_70x90mm_31x26-prt329.ipt
- C:\Users\Vincent Larson\Downloads\Universal_board_70x90mm_31x26\Universal_board_70x90mm_31x26-prt330.ipt
- C:\Users\Vincent Larson\Downloads\Universal_board_70x90mm_31x26\Universal_board_70x90mm_31x26-prt331.ipt
- C:\Users\Vincent Larson\Downloads\Universal_board_70x90mm_31x26\Universal_board_70x90mm_31x26-prt332.ipt
- C:\Users\Vincent Larson\Downloads\Universal_board_70x90mm_31x26\Universal_board_70x90mm_31x26-prt333.ipt
- C:\Users\Vincent Larson\Downloads\Universal_board_70x90mm_31x26\Universal_board_70x90mm_31x26-prt334.ipt
- C:\Users\Vincent Larson\Downloads\Universal_board_70x90mm_31x26\Universal_board_70x90mm_31x26-prt335.ipt
- C:\Users\Vincent Larson\Downloads\Universal_board_70x90mm_31x26\Universal_board_70x90mm_31x26-prt336.ipt
- C:\Users\Vincent Larson\Downloads\Universal_board_70x90mm_31x26\Universal_board_70x90mm_31x26-prt337.ipt
- C:\Users\Vincent Larson\Downloads\Universal_board_70x90mm_31x26\Universal_board_70x90mm_31x26-prt338.ipt
- C:\Users\Vincent Larson\Downloads\Universal_board_70x90mm_31x26\Universal_board_70x90mm_31x26-prt339.ipt
- C:\Users\Vincent Larson\Downloads\Universal_board_70x90mm_31x26\Universal_board_70x90mm_31x26-prt340.ipt
- C:\Users\Vincent Larson\Downloads\Universal_board_70x90mm_31x26\Universal_board_70x90mm_31x26-prt341.ipt
- C:\Users\Vincent Larson\Downloads\Universal_board_70x90mm_31x26\Universal_board_70x90mm_31x26-prt342.ipt
- C:\Users\Vincent Larson\Downloads\Universal_board_70x90mm_31x26\Universal_board_70x90mm_31x26-prt343.ipt
- C:\Users\Vincent Larson\Downloads\Universal_board_70x90mm_31x26\Universal_board_70x90mm_31x26-prt344.ipt
- C:\Users\Vincent Larson\Downloads\Universal_board_70x90mm_31x26\Universal_board_70x90mm_31x26-prt345.ipt
- C:\Users\Vincent Larson\Downloads\Universal_board_70x90mm_31x26\Universal_board_70x90mm_31x26-prt346.ipt
- C:\Users\Vincent Larson\Downloads\Universal_board_70x90mm_31x26\Universal_board_70x90mm_31x26-prt347.ipt
- C:\Users\Vincent Larson\Downloads\Universal_board_70x90mm_31x26\Universal_board_70x90mm_31x26-prt348.ipt
- C:\Users\Vincent Larson\Downloads\Universal_board_70x90mm_31x26\Universal_board_70x90mm_31x26-prt349.ipt
- C:\Users\Vincent Larson\Downloads\Universal_board_70x90mm_31x26\Universal_board_70x90mm_31x26-prt350.ipt
- C:\Users\Vincent Larson\Downloads\Universal_board_70x90mm_31x26\Universal_board_70x90mm_31x26-prt351.ipt
- C:\Users\Vincent Larson\Downloads\Universal_board_70x90mm_31x26\Universal_board_70x90mm_31x26-prt352.ipt
- C:\Users\Vincent Larson\Downloads\Universal_board_70x90mm_31x26\Universal_board_70x90mm_31x26-prt353.ipt
- C:\Users\Vincent Larson\Downloads\Universal_board_70x90mm_31x26\Universal_board_70x90mm_31x26-prt354.ipt
- C:\Users\Vincent Larson\Downloads\Universal_board_70x90mm_31x26\Universal_board_70x90mm_31x26-prt355.ipt
- C:\Users\Vincent Larson\Downloads\Universal_board_70x90mm_31x26\Universal_board_70x90mm_31x26-prt356.ipt
- C:\Users\Vincent Larson\Downloads\Universal_board_70x90mm_31x26\Universal_board_70x90mm_31x26-prt357.ipt
- C:\Users\Vincent Larson\Downloads\Universal_board_70x90mm_31x26\Universal_board_70x90mm_31x26-prt358.ipt
- C:\Users\Vincent Larson\Downloads\Universal_board_70x90mm_31x26\Universal_board_70x90mm_31x26-prt359.ipt
- C:\Users\Vincent Larson\Downloads\Universal_board_70x90mm_31x26\Universal_board_70x90mm_31x26-prt360.ipt
- C:\Users\Vincent Larson\Downloads\Universal_board_70x90mm_31x26\Universal_board_70x90mm_31x26-prt361.ipt
- C:\Users\Vincent Larson\Downloads\Universal_board_70x90mm_31x26\Universal_board_70x90mm_31x26-prt362.ipt
- C:\Users\Vincent Larson\Downloads\Universal_board_70x90mm_31x26\Universal_board_70x90mm_31x26-prt363.ipt
- C:\Users\Vincent Larson\Downloads\Universal_board_70x90mm_31x26\Universal_board_70x90mm_31x26-prt364.ipt
- C:\Users\Vincent Larson\Downloads\Universal_board_70x90mm_31x26\Universal_board_70x90mm_31x26-prt365.ipt
- C:\Users\Vincent Larson\Downloads\Universal_board_70x90mm_31x26\Universal_board_70x90mm_31x26-prt366.ipt
- C:\Users\Vincent Larson\Downloads\Universal_board_70x90mm_31x26\Universal_board_70x90mm_31x26-prt367.ipt
- C:\Users\Vincent Larson\Downloads\Universal_board_70x90mm_31x26\Universal_board_70x90mm_31x26-prt368.ipt
- C:\Users\Vincent Larson\Downloads\Universal_board_70x90mm_31x26\Universal_board_70x90mm_31x26-prt369.ipt
- C:\Users\Vincent Larson\Downloads\Universal_board_70x90mm_31x26\Universal_board_70x90mm_31x26-prt370.ipt
- C:\Users\Vincent Larson\Downloads\Universal_board_70x90mm_31x26\Universal_board_70x90mm_31x26-prt371.ipt
- C:\Users\Vincent Larson\Downloads\Universal_board_70x90mm_31x26\Universal_board_70x90mm_31x26-prt372.ipt
- C:\Users\Vincent Larson\Downloads\Universal_board_70x90mm_31x26\Universal_board_70x90mm_31x26-prt373.ipt
- C:\Users\Vincent Larson\Downloads\Universal_board_70x90mm_31x26\Universal_board_70x90mm_31x26-prt374.ipt
- C:\Users\Vincent Larson\Downloads\Universal_board_70x90mm_31x26\Universal_board_70x90mm_31x26-prt375.ipt
- C:\Users\Vincent Larson\Downloads\Universal_board_70x90mm_31x26\Universal_board_70x90mm_31x26-prt376.ipt
- C:\Users\Vincent Larson\Downloads\Universal_board_70x90mm_31x26\Universal_board_70x90mm_31x26-prt377.ipt
- C:\Users\Vincent Larson\Downloads\Universal_board_70x90mm_31x26\Universal_board_70x90mm_31x26-prt378.ipt
- C:\Users\Vincent Larson\Downloads\Universal_board_70x90mm_31x26\Universal_board_70x90mm_31x26-prt379.ipt
- C:\Users\Vincent Larson\Downloads\Universal_board_70x90mm_31x26\Universal_board_70x90mm_31x26-prt380.ipt
- C:\Users\Vincent Larson\Downloads\Universal_board_70x90mm_31x26\Universal_board_70x90mm_31x26-prt381.ipt
- C:\Users\Vincent Larson\Downloads\Universal_board_70x90mm_31x26\Universal_board_70x90mm_31x26-prt382.ipt
- C:\Users\Vincent Larson\Downloads\Universal_board_70x90mm_31x26\Universal_board_70x90mm_31x26-prt383.ipt
- C:\Users\Vincent Larson\Downloads\Universal_board_70x90mm_31x26\Universal_board_70x90mm_31x26-prt384.ipt
- C:\Users\Vincent Larson\Downloads\Universal_board_70x90mm_31x26\Universal_board_70x90mm_31x26-prt385.ipt
- C:\Users\Vincent Larson\Downloads\Universal_board_70x90mm_31x26\Universal_board_70x90mm_31x26-prt386.ipt
- C:\Users\Vincent Larson\Downloads\Universal_board_70x90mm_31x26\Universal_board_70x90mm_31x26-prt387.ipt
- C:\Users\Vincent Larson\Downloads\Universal_board_70x90mm_31x26\Universal_board_70x90mm_31x26-prt388.ipt
- C:\Users\Vincent Larson\Downloads\Universal_board_70x90mm_31x26\Universal_board_70x90mm_31x26-prt389.ipt
- C:\Users\Vincent Larson\Downloads\Universal_board_70x90mm_31x26\Universal_board_70x90mm_31x26-prt390.ipt
- C:\Users\Vincent Larson\Downloads\Universal_board_70x90mm_31x26\Universal_board_70x90mm_31x26-prt391.ipt
- C:\Users\Vincent Larson\Downloads\Universal_board_70x90mm_31x26\Universal_board_70x90mm_31x26-prt392.ipt
- C:\Users\Vincent Larson\Downloads\Universal_board_70x90mm_31x26\Universal_board_70x90mm_31x26-prt393.ipt
- C:\Users\Vincent Larson\Downloads\Universal_board_70x90mm_31x26\Universal_board_70x90mm_31x26-prt394.ipt
- C:\Users\Vincent Larson\Downloads\Universal_board_70x90mm_31x26\Universal_board_70x90mm_31x26-prt395.ipt
- C:\Users\Vincent Larson\Downloads\Universal_board_70x90mm_31x26\Universal_board_70x90mm_31x26-prt396.ipt
- C:\Users\Vincent Larson\Downloads\Universal_board_70x90mm_31x26\Universal_board_70x90mm_31x26-prt397.ipt
- C:\Users\Vincent Larson\Downloads\Universal_board_70x90mm_31x26\Universal_board_70x90mm_31x26-prt398.ipt
- C:\Users\Vincent Larson\Downloads\Universal_board_70x90mm_31x26\Universal_board_70x90mm_31x26-prt399.ipt
- C:\Users\Vincent Larson\Downloads\Universal_board_70x90mm_31x26\Universal_board_70x90mm_31x26-prt400.ipt
- C:\Users\Vincent Larson\Downloads\Universal_board_70x90mm_31x26\Universal_board_70x90mm_31x26-prt401.ipt
- C:\Users\Vincent Larson\Downloads\Universal_board_70x90mm_31x26\Universal_board_70x90mm_31x26-prt402.ipt
- C:\Users\Vincent Larson\Downloads\Universal_board_70x90mm_31x26\Universal_board_70x90mm_31x26-prt403.ipt
- C:\Users\Vincent Larson\Downloads\Universal_board_70x90mm_31x26\Universal_board_70x90mm_31x26-prt404.ipt
- C:\Users\Vincent Larson\Downloads\Universal_board_70x90mm_31x26\Universal_board_70x90mm_31x26-prt405.ipt
- C:\Users\Vincent Larson\Downloads\Universal_board_70x90mm_31x26\Universal_board_70x90mm_31x26-prt406.ipt
- C:\Users\Vincent Larson\Downloads\Universal_board_70x90mm_31x26\Universal_board_70x90mm_31x26-prt407.ipt
- C:\Users\Vincent Larson\Downloads\Universal_board_70x90mm_31x26\Universal_board_70x90mm_31x26-prt408.ipt
- C:\Users\Vincent Larson\Downloads\Universal_board_70x90mm_31x26\Universal_board_70x90mm_31x26-prt409.ipt
- C:\Users\Vincent Larson\Downloads\Universal_board_70x90mm_31x26\Universal_board_70x90mm_31x26-prt410.ipt
- C:\Users\Vincent Larson\Downloads\Universal_board_70x90mm_31x26\Universal_board_70x90mm_31x26-prt411.ipt
- C:\Users\Vincent Larson\Downloads\Universal_board_70x90mm_31x26\Universal_board_70x90mm_31x26-prt412.ipt
- C:\Users\Vincent Larson\Downloads\Universal_board_70x90mm_31x26\Universal_board_70x90mm_31x26-prt413.ipt
- C:\Users\Vincent Larson\Downloads\Universal_board_70x90mm_31x26\Universal_board_70x90mm_31x26-prt414.ipt
- C:\Users\Vincent Larson\Downloads\Universal_board_70x90mm_31x26\Universal_board_70x90mm_31x26-prt415.ipt
- C:\Users\Vincent Larson\Downloads\Universal_board_70x90mm_31x26\Universal_board_70x90mm_31x26-prt416.ipt
- C:\Users\Vincent Larson\Downloads\Universal_board_70x90mm_31x26\Universal_board_70x90mm_31x26-prt417.ipt
- C:\Users\Vincent Larson\Downloads\Universal_board_70x90mm_31x26\Universal_board_70x90mm_31x26-prt418.ipt
- C:\Users\Vincent Larson\Downloads\Universal_board_70x90mm_31x26\Universal_board_70x90mm_31x26-prt419.ipt
- C:\Users\Vincent Larson\Downloads\Universal_board_70x90mm_31x26\Universal_board_70x90mm_31x26-prt420.ipt
- C:\Users\Vincent Larson\Downloads\Universal_board_70x90mm_31x26\Universal_board_70x90mm_31x26-prt421.ipt
- C:\Users\Vincent Larson\Downloads\Universal_board_70x90mm_31x26\Universal_board_70x90mm_31x26-prt422.ipt
- C:\Users\Vincent Larson\Downloads\Universal_board_70x90mm_31x26\Universal_board_70x90mm_31x26-prt423.ipt
- C:\Users\Vincent Larson\Downloads\Universal_board_70x90mm_31x26\Universal_board_70x90mm_31x26-prt424.ipt
- C:\Users\Vincent Larson\Downloads\Universal_board_70x90mm_31x26\Universal_board_70x90mm_31x26-prt425.ipt
- C:\Users\Vincent Larson\Downloads\Universal_board_70x90mm_31x26\Universal_board_70x90mm_31x26-prt426.ipt
- C:\Users\Vincent Larson\Downloads\Universal_board_70x90mm_31x26\Universal_board_70x90mm_31x26-prt427.ipt
- C:\Users\Vincent Larson\Downloads\Universal_board_70x90mm_31x26\Universal_board_70x90mm_31x26-prt428.ipt
- C:\Users\Vincent Larson\Downloads\Universal_board_70x90mm_31x26\Universal_board_70x90mm_31x26-prt429.ipt
- C:\Users\Vincent Larson\Downloads\Universal_board_70x90mm_31x26\Universal_board_70x90mm_31x26-prt430.ipt
- C:\Users\Vincent Larson\Downloads\Universal_board_70x90mm_31x26\Universal_board_70x90mm_31x26-prt431.ipt
- C:\Users\Vincent Larson\Downloads\Universal_board_70x90mm_31x26\Universal_board_70x90mm_31x26-prt432.ipt
- C:\Users\Vincent Larson\Downloads\Universal_board_70x90mm_31x26\Universal_board_70x90mm_31x26-prt433.ipt
- C:\Users\Vincent Larson\Downloads\Universal_board_70x90mm_31x26\Universal_board_70x90mm_31x26-prt434.ipt
- C:\Users\Vincent Larson\Downloads\Universal_board_70x90mm_31x26\Universal_board_70x90mm_31x26-prt435.ipt
- C:\Users\Vincent Larson\Downloads\Universal_board_70x90mm_31x26\Universal_board_70x90mm_31x26-prt436.ipt
- C:\Users\Vincent Larson\Downloads\Universal_board_70x90mm_31x26\Universal_board_70x90mm_31x26-prt437.ipt
- C:\Users\Vincent Larson\Downloads\Universal_board_70x90mm_31x26\Universal_board_70x90mm_31x26-prt438.ipt
- C:\Users\Vincent Larson\Downloads\Universal_board_70x90mm_31x26\Universal_board_70x90mm_31x26-prt439.ipt
- C:\Users\Vincent Larson\Downloads\Universal_board_70x90mm_31x26\Universal_board_70x90mm_31x26-prt440.ipt
- C:\Users\Vincent Larson\Downloads\Universal_board_70x90mm_31x26\Universal_board_70x90mm_31x26-prt441.ipt
- C:\Users\Vincent Larson\Downloads\Universal_board_70x90mm_31x26\Universal_board_70x90mm_31x26-prt442.ipt
- C:\Users\Vincent Larson\Downloads\Universal_board_70x90mm_31x26\Universal_board_70x90mm_31x26-prt443.ipt
- C:\Users\Vincent Larson\Downloads\Universal_board_70x90mm_31x26\Universal_board_70x90mm_31x26-prt444.ipt
- C:\Users\Vincent Larson\Downloads\Universal_board_70x90mm_31x26\Universal_board_70x90mm_31x26-prt445.ipt
- C:\Users\Vincent Larson\Downloads\Universal_board_70x90mm_31x26\Universal_board_70x90mm_31x26-prt446.ipt
- C:\Users\Vincent Larson\Downloads\Universal_board_70x90mm_31x26\Universal_board_70x90mm_31x26-prt447.ipt
- C:\Users\Vincent Larson\Downloads\Universal_board_70x90mm_31x26\Universal_board_70x90mm_31x26-prt448.ipt
- C:\Users\Vincent Larson\Downloads\Universal_board_70x90mm_31x26\Universal_board_70x90mm_31x26-prt449.ipt
- C:\Users\Vincent Larson\Downloads\Universal_board_70x90mm_31x26\Universal_board_70x90mm_31x26-prt450.ipt
- C:\Users\Vincent Larson\Downloads\Universal_board_70x90mm_31x26\Universal_board_70x90mm_31x26-prt451.ipt
- C:\Users\Vincent Larson\Downloads\Universal_board_70x90mm_31x26\Universal_board_70x90mm_31x26-prt452.ipt
- C:\Users\Vincent Larson\Downloads\Universal_board_70x90mm_31x26\Universal_board_70x90mm_31x26-prt453.ipt
- C:\Users\Vincent Larson\Downloads\Universal_board_70x90mm_31x26\Universal_board_70x90mm_31x26-prt454.ipt
- C:\Users\Vincent Larson\Downloads\Universal_board_70x90mm_31x26\Universal_board_70x90mm_31x26-prt455.ipt
- C:\Users\Vincent Larson\Downloads\Universal_board_70x90mm_31x26\Universal_board_70x90mm_31x26-prt456.ipt
- C:\Users\Vincent Larson\Downloads\Universal_board_70x90mm_31x26\Universal_board_70x90mm_31x26-prt457.ipt
- C:\Users\Vincent Larson\Downloads\Universal_board_70x90mm_31x26\Universal_board_70x90mm_31x26-prt458.ipt
- C:\Users\Vincent Larson\Downloads\Universal_board_70x90mm_31x26\Universal_board_70x90mm_31x26-prt459.ipt
- C:\Users\Vincent Larson\Downloads\Universal_board_70x90mm_31x26\Universal_board_70x90mm_31x26-prt460.ipt